# Autodesk Inventor assembly: Cover Assembly Vibrometer
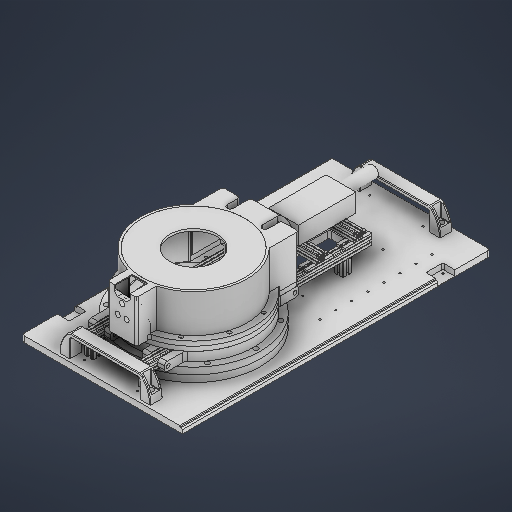
[picture p0: Inventor's stored thumbnail of the model, 512x512]
Saved by Autodesk Inventor 2025 (Build 290162000, 162)
## iProperties
Created: 2025-03-28
Part Number: Cover Assembly Vibrometer
Document SubType Name: Assembly
Designer: mayhe
Author: mayhe
## Documents named in this file (14)
- C:\Users\mayhe\OneDrive\Documents\In-situ-monitoring-of-powder-bed-fusion-additive-manufacturing\system_development\Orichalcum\v0.2\Hardware_design\custom-cover\Cover Assembly Vibrometer.iam
- C:\Users\mayhe\OneDrive\Documents\In-situ-monitoring-of-powder-bed-fusion-additive-manufacturing\system_development\Orichalcum\v0.2\Hardware_design\custom-cover\cover\Updated Cover (Vibrometer).ipt
- C:\Users\mayhe\OneDrive\Documents\In-situ-monitoring-of-powder-bed-fusion-additive-manufacturing\system_development\Mithril\v0.2\Model\300mm Housing 1.ipt
- C:\Users\mayhe\OneDrive\Documents\In-situ-monitoring-of-powder-bed-fusion-additive-manufacturing\system_development\Mithril\v0.2\Model\300mm housing 2 Camera.ipt
- C:\Users\mayhe\OneDrive\Documents\In-situ-monitoring-of-powder-bed-fusion-additive-manufacturing\system_development\Orichalcum\v0.2\Hardware_design\custom-cover\cylinder-parts\Cylinder 80-20 Spacer_2.ipt
- C:\Users\mayhe\OneDrive\Documents\In-situ-monitoring-of-powder-bed-fusion-additive-manufacturing\system_development\Orichalcum\v0.2\Hardware_design\custom-cover\cylinder-parts\Cylinder 80-20 Spacer_1.ipt
- C:\Users\mayhe\OneDrive\Documents\In-situ-monitoring-of-powder-bed-fusion-additive-manufacturing\system_development\Orichalcum\v0.2\Hardware_design\custom-cover\8020-parts\20-2020-500-CL.ipt
- C:\Users\mayhe\OneDrive\Documents\In-situ-monitoring-of-powder-bed-fusion-additive-manufacturing\system_development\Orichalcum\v0.2\Hardware_design\custom-cover\813RC8_AF0.ipt
- C:\Users\mayhe\OneDrive\Documents\In-situ-monitoring-of-powder-bed-fusion-additive-manufacturing\system_development\Orichalcum\v0.2\Hardware_design\custom-cover\8020-parts\20-2020-30-CL.ipt
- C:\Users\mayhe\OneDrive\Documents\In-situ-monitoring-of-powder-bed-fusion-additive-manufacturing\system_development\Orichalcum\v0.2\Hardware_design\custom-cover\cover\Spacer Laser.ipt
- C:\Users\mayhe\OneDrive\Documents\In-situ-monitoring-of-powder-bed-fusion-additive-manufacturing\system_development\Orichalcum\v0.2\Hardware_design\custom-cover\cylinder-parts\cylinder-segments\Cylinder Segment  Camera + Galvo.ipt
- C:\Users\mayhe\OneDrive\Documents\In-situ-monitoring-of-powder-bed-fusion-additive-manufacturing\system_development\Orichalcum\v0.2\Hardware_design\custom-cover\cylinder-parts\final-parts\Cylinder Slidey Bit Housing Camera + galvo.ipt
- C:\Users\mayhe\OneDrive\Documents\In-situ-monitoring-of-powder-bed-fusion-additive-manufacturing\system_development\Orichalcum\v0.2\Hardware_design\custom-cover\8020-parts\20-2020-140_25-CL.ipt
- C:\Users\mayhe\OneDrive\Documents\In-situ-monitoring-of-powder-bed-fusion-additive-manufacturing\system_development\Orichalcum\v0.2\Hardware_design\laser-vibrometer\Updated Laser Scanner.ipt
## Components (24 placed, 13 different names)
1. Updated Cover (Vibrometer):1 — Rotational:1, Rotational:7, Rotational:8, Rotational:9, Rigid:1, Rotational:14, Rotational:15
2. 300mm Housing 1:1 — Rotational:1, Rotational:2
3. 300mm housing 2 Camera:1 — Rotational:2, Rotational:3, Rotational:4, Rotational:5, Rotational:6, Mate:1, Mate:4
4. Cylinder 80-20 Spacer_2:1 — Rotational:3, Flush:2, Mate:3
5. Cylinder 80-20 Spacer_2:2 — Rotational:4, Flush:1, Mate:2, Rotational:13
6. Cylinder 80-20 Spacer_1:1 — Rotational:5
7. Cylinder 80-20 Spacer_1:2 — Rotational:6
8. 20-2020-500-CL:1 — Flush:2, Mate:3, Mate:4, Mate:6, Flush:5, Flush:6, Mate:13, Flush:12
9. 20-2020-500-CL:2 — Flush:1, Mate:1, Mate:2, Mate:5, Flush:3, Flush:4, Flush:9, Mate:12, Flush:10
10. 813RC8_AF0:1 — Rotational:7
11. 813RC8_AF0:2 — Rotational:8
12. 20-2020-30-CL:1 — Rotational:9
13. 20-2020-30-CL:2 — Rigid:1
14. Spacer Laser:1 — Mate:13, Flush:12, Flush:13
15. Spacer Laser:2 — Mate:6, Flush:5, Flush:6
16. 20-2020-140_25-CL:1 — Mate:10, Flush:9, Mate:11, Flush:11, Flush:13
17. 20-2020-140_25-CL:2 — Mate:7, Flush:7, Flush:8, Mate:8, Mate:9
18. Spacer Laser:3 — Mate:5, Flush:3, Flush:4, Mate:7, Flush:7, Flush:8
19. Spacer Laser:4 — Mate:12, Flush:10, Flush:11
20. Cylinder Slidey Bit Housing Camera + galvo:1 — Rotational:12
21. Cylinder Segment  Camera + Galvo:1 — Rotational:12, Rotational:13
22. Updated Laser Scanner:1 — Mate:8, Mate:9, Mate:10, Mate:11
23. 20-2020-30-CL:3 — Rotational:15
24. 20-2020-30-CL:4 — Rotational:14
## Relationships (40: RevoluteJoint 13, Flush 13, Mate 13, WeldJoint 1)
- Rotational:1 [RevoluteJoint]: Updated Cover (Vibrometer):1 ↔ 300mm Housing 1:1
- Rotational:2 [RevoluteJoint]: 300mm Housing 1:1 ↔ 300mm housing 2 Camera:1
- Rotational:3 [RevoluteJoint]: 300mm housing 2 Camera:1 ↔ Cylinder 80-20 Spacer_2:1
- Rotational:4 [RevoluteJoint]: 300mm housing 2 Camera:1 ↔ Cylinder 80-20 Spacer_2:2
- Rotational:5 [RevoluteJoint]: 300mm housing 2 Camera:1 ↔ Cylinder 80-20 Spacer_1:1
- Rotational:6 [RevoluteJoint]: 300mm housing 2 Camera:1 ↔ Cylinder 80-20 Spacer_1:2
- Flush:1 (-20 mm): Cylinder 80-20 Spacer_2:2 ↔ 20-2020-500-CL:2
- Mate:1: 300mm housing 2 Camera:1 ↔ 20-2020-500-CL:2
- Mate:2: Cylinder 80-20 Spacer_2:2 ↔ 20-2020-500-CL:2
- Flush:2 (-20 mm): Cylinder 80-20 Spacer_2:1 ↔ 20-2020-500-CL:1
- Rotational:7 [RevoluteJoint]: Updated Cover (Vibrometer):1 ↔ 813RC8_AF0:1
- Rotational:8 [RevoluteJoint]: Updated Cover (Vibrometer):1 ↔ 813RC8_AF0:2
- Rotational:9 [RevoluteJoint]: Updated Cover (Vibrometer):1 ↔ 20-2020-30-CL:1
- Rigid:1 [WeldJoint]: Updated Cover (Vibrometer):1 ↔ 20-2020-30-CL:2
- Mate:3: Cylinder 80-20 Spacer_2:1 ↔ 20-2020-500-CL:1
- Mate:4: 300mm housing 2 Camera:1 ↔ 20-2020-500-CL:1
- Mate:5: 20-2020-500-CL:2 ↔ Spacer Laser:3
- Flush:3: 20-2020-500-CL:2 ↔ Spacer Laser:3
- Flush:4: 20-2020-500-CL:2 ↔ Spacer Laser:3
- Mate:6: 20-2020-500-CL:1 ↔ Spacer Laser:2
- Flush:5: 20-2020-500-CL:1 ↔ Spacer Laser:2
- Flush:6: 20-2020-500-CL:1 ↔ Spacer Laser:2
- Mate:7: 20-2020-140_25-CL:2 ↔ Spacer Laser:3
- Flush:7: 20-2020-140_25-CL:2 ↔ Spacer Laser:3
- Flush:8 (20 mm): 20-2020-140_25-CL:2 ↔ Spacer Laser:3
- Rotational:12 [RevoluteJoint]: Cylinder Slidey Bit Housing Camera + galvo:1 ↔ Cylinder Segment  Camera + Galvo:1
- Mate:8: 20-2020-140_25-CL:2 ↔ Updated Laser Scanner:1
- Mate:9: 20-2020-140_25-CL:2 ↔ Updated Laser Scanner:1
- Rotational:13 [RevoluteJoint]: Cylinder 80-20 Spacer_2:2 ↔ Cylinder Segment  Camera + Galvo:1
- Mate:10: 20-2020-140_25-CL:1 ↔ Updated Laser Scanner:1
- Flush:9: 20-2020-500-CL:2 ↔ 20-2020-140_25-CL:1
- Mate:11: 20-2020-140_25-CL:1 ↔ Updated Laser Scanner:1
- Mate:12: 20-2020-500-CL:2 ↔ Spacer Laser:4
- Flush:10: 20-2020-500-CL:2 ↔ Spacer Laser:4
- Flush:11 (-20 mm): 20-2020-140_25-CL:1 ↔ Spacer Laser:4
- Mate:13: 20-2020-500-CL:1 ↔ Spacer Laser:1
- Flush:12: 20-2020-500-CL:1 ↔ Spacer Laser:1
- Flush:13 (-20 mm): Spacer Laser:1 ↔ 20-2020-140_25-CL:1
- Rotational:14 [RevoluteJoint]: Updated Cover (Vibrometer):1 ↔ 20-2020-30-CL:4
- Rotational:15 [RevoluteJoint]: Updated Cover (Vibrometer):1 ↔ 20-2020-30-CL:3
